# Autodesk Inventor assembly: Manifold
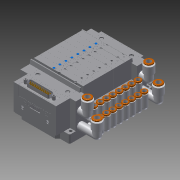
[picture p0: Inventor's stored thumbnail of the model, 180x180]
Saved by Autodesk Inventor 2014 (Build 180170000, 170)
## iProperties
Created: 2014-01-20
Part Number: Manifold
Document SubType Name: Assembly
Designer: Andrew Toennies
Author: Andrew Toennies
## Documents named in this file (36)
- C:\Users\Andrew Toennies\Documents\GitHub\2014buildCAD\New Shooter\Manifold and Valves\Manifold.iam
- C:\Users\Andrew Toennies\Documents\GitHub\2014buildCAD\Imported Components\SS5Y3-10F1-08B-LN7\Part70.ipt
- C:\Users\Andrew Toennies\Documents\GitHub\2014buildCAD\Imported Components\SS5Y3-10F1-08B-LN7\Part72.ipt
- C:\Users\Andrew Toennies\Documents\GitHub\2014buildCAD\Imported Components\SS5Y3-10F1-08B-LN7\Part74.ipt
- C:\Users\Andrew Toennies\Documents\GitHub\2014buildCAD\Imported Components\SS5Y3-10F1-08B-LN7\Part76.ipt
- C:\Users\Andrew Toennies\Documents\GitHub\2014buildCAD\Imported Components\SS5Y3-10F1-08B-LN7\Part78.ipt
- C:\Users\Andrew Toennies\Documents\GitHub\2014buildCAD\Imported Components\SS5Y3-10F1-08B-LN7\Part80.ipt
- C:\Users\Andrew Toennies\Documents\GitHub\2014buildCAD\Imported Components\SS5Y3-10F1-08B-LN7\Part82.ipt
- C:\Users\Andrew Toennies\Documents\GitHub\2014buildCAD\Imported Components\SS5Y3-10F1-08B-LN7\Part84.ipt
- C:\Users\Andrew Toennies\Documents\GitHub\2014buildCAD\Imported Components\SS5Y3-10F1-08B-LN7\Part86.ipt
- C:\Users\Andrew Toennies\Documents\GitHub\2014buildCAD\Imported Components\SS5Y3-10F1-08B-LN7\Part88.ipt
- C:\Users\Andrew Toennies\Documents\GitHub\2014buildCAD\Imported Components\SS5Y3-10F1-08B-LN7\Part90.ipt
- C:\Users\Andrew Toennies\Documents\GitHub\2014buildCAD\Imported Components\SS5Y3-10F1-08B-LN7\Part92.ipt
- C:\Users\Andrew Toennies\Documents\GitHub\2014buildCAD\Imported Components\SS5Y3-10F1-08B-LN7\Part94.ipt
- C:\Users\Andrew Toennies\Documents\GitHub\2014buildCAD\Imported Components\SS5Y3-10F1-08B-LN7\Part96.ipt
- C:\Users\Andrew Toennies\Documents\GitHub\2014buildCAD\Imported Components\SS5Y3-10F1-08B-LN7\Part98.ipt
- C:\Users\Andrew Toennies\Documents\GitHub\2014buildCAD\Imported Components\SS5Y3-10F1-08B-LN7\Part100.ipt
- C:\Users\Andrew Toennies\Documents\GitHub\2014buildCAD\Imported Components\SS5Y3-10F1-08B-LN7\Part102.ipt
- C:\Users\Andrew Toennies\Documents\GitHub\2014buildCAD\Imported Components\SS5Y3-10F1-08B-LN7\Part104.ipt
- C:\Users\Andrew Toennies\Documents\GitHub\2014buildCAD\Imported Components\SS5Y3-10F1-08B-LN7\Part106.ipt
- C:\Users\Andrew Toennies\Documents\GitHub\2014buildCAD\Imported Components\SS5Y3-10F1-08B-LN7\Part108.ipt
- C:\Users\Andrew Toennies\Documents\GitHub\2014buildCAD\Imported Components\SS5Y3-10F1-08B-LN7\Part110.ipt
- C:\Users\Andrew Toennies\Documents\GitHub\2014buildCAD\Imported Components\SS5Y3-10F1-08B-LN7\Part112.ipt
- C:\Users\Andrew Toennies\Documents\GitHub\2014buildCAD\Imported Components\SS5Y3-10F1-08B-LN7\Part114.ipt
- C:\Users\Andrew Toennies\Documents\GitHub\2014buildCAD\Imported Components\SS5Y3-10F1-08B-LN7\Part116.ipt
- C:\Users\Andrew Toennies\Documents\GitHub\2014buildCAD\Imported Components\SS5Y3-10F1-08B-LN7\Part118.ipt
- C:\Users\Andrew Toennies\Documents\GitHub\2014buildCAD\Imported Components\SS5Y3-10F1-08B-LN7\Part120.ipt
- C:\Users\Andrew Toennies\Documents\GitHub\2014buildCAD\Imported Components\SS5Y3-10F1-08B-LN7\Part122.ipt
- C:\Users\Andrew Toennies\Documents\GitHub\2014buildCAD\Imported Components\SS5Y3-10F1-08B-LN7\Part124.ipt
- C:\Users\Andrew Toennies\Documents\GitHub\2014buildCAD\Imported Components\SS5Y3-10F1-08B-LN7\Part126.ipt
- C:\Users\Andrew Toennies\Documents\GitHub\2014buildCAD\Imported Components\SS5Y3-10F1-08B-LN7\Part128.ipt
- C:\Users\Andrew Toennies\Documents\GitHub\2014buildCAD\Imported Components\SS5Y3-10F1-08B-LN7\Part130.ipt
- C:\Users\Andrew Toennies\Documents\GitHub\2014buildCAD\Imported Components\SS5Y3-10F1-08B-LN7\Part132.ipt
- C:\Users\Andrew Toennies\Documents\GitHub\2014buildCAD\Imported Components\SS5Y3-10F1-08B-LN7\Part134.ipt
- C:\Users\Andrew Toennies\Documents\GitHub\2014buildCAD\Imported Components\SS5Y3-10F1-08B-LN7\Part136.ipt
- C:\Users\Andrew Toennies\Documents\GitHub\2014buildCAD\New Shooter\Manifold and Valves\Valve.iam
## Components (42 placed, 35 different names)
1. Part70:1
2. Part72:1
3. Part74:1
4. Part76:1 — Mate:1, Flush:3
5. Part78:1
6. Part80:1
7. Part82:1
8. Part84:1
9. Part86:1
10. Part88:1
11. Part90:1 — Mate:16
12. Part92:1 — Mate:14
13. Part94:1 — Mate:12
14. Part96:1 — Mate:10
15. Part98:1 — Mate:8
16. Part100:1 — Mate:6
17. Part102:1 — Mate:2, Mate:4
18. Part104:1
19. Part106:1
20. Part108:1
21. Part110:1
22. Part112:1
23. Part114:1
24. Part116:1
25. Part118:1
26. Part120:1
27. Part122:1
28. Part124:1
29. Part126:1
30. Part128:1
31. Part130:1
32. Part132:1
33. Part134:1
34. Part136:1
35. Valve:1 [sub-assembly] — Mate:5, Mate:6, Flush:2, Mate:7
36. Valve:2 [sub-assembly] — Mate:1, Mate:2, Mate:3, Flush:1, Flush:3
37. Valve:3 [sub-assembly] — Mate:7, Mate:8, Flush:4, Mate:9, Flush:5
38. Valve:4 [sub-assembly] — Mate:11, Flush:6, Mate:12, Mate:13, Flush:7
39. Valve:5 [sub-assembly] — Mate:13, Flush:7, Mate:14, Mate:15, Flush:8
40. Valve:6 [sub-assembly] — Mate:15, Flush:8, Mate:16
41. Valve:7 [sub-assembly] — Mate:9, Flush:5, Mate:10, Mate:11, Flush:6
42. Valve:8 [sub-assembly] — Mate:3, Mate:4, Mate:5, Flush:1, Flush:2, Flush:4
## Relationships (24: Mate 16, Flush 8)
- Mate:1: Part76:1 ↔ Valve:2
- Mate:2: Part102:1 ↔ Valve:2
- Mate:3: Valve:2 ↔ Valve:8
- Mate:4: Part102:1 ↔ Valve:8
- Mate:5: Valve:1 ↔ Valve:8
- Mate:6: Part100:1 ↔ Valve:1
- Flush:1: Valve:2 ↔ Valve:8
- Flush:2: Valve:1 ↔ Valve:8
- Flush:3: Part76:1 ↔ Valve:2
- Mate:7: Valve:1 ↔ Valve:3
- Mate:8: Part98:1 ↔ Valve:3
- Flush:4: Valve:3 ↔ Valve:8
- Mate:9: Valve:3 ↔ Valve:7
- Flush:5: Valve:3 ↔ Valve:7
- Mate:10: Part96:1 ↔ Valve:7
- Mate:11: Valve:4 ↔ Valve:7
- Flush:6: Valve:4 ↔ Valve:7
- Mate:12: Part94:1 ↔ Valve:4
- Mate:13: Valve:4 ↔ Valve:5
- Flush:7: Valve:4 ↔ Valve:5
- Mate:14: Part92:1 ↔ Valve:5
- Mate:15: Valve:5 ↔ Valve:6
- Flush:8: Valve:5 ↔ Valve:6
- Mate:16: Part90:1 ↔ Valve:6
